# Autodesk Inventor assembly: Stator_Assembly_2_0_2
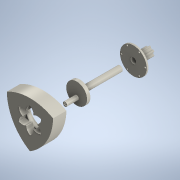
[picture p0: Inventor's stored thumbnail of the model, 180x180]
Saved by Autodesk Inventor 2021 (Build 250183000, 183)
## iProperties
Created: 2021-04-19
Part Number: Stator_Assembly_2_0_2
Document SubType Name: Assembly
Designer: lucia
Author: lucia
## Documents named in this file (4)
- E:\Documents\Inventor\Fixed Rotor Wankel Engine\Assemblies\Stator_Assembly_2_0_2.iam
- E:\Documents\Inventor\Fixed Rotor Wankel Engine\Parts\Rotor_Mount.ipt
- E:\Documents\Inventor\Fixed Rotor Wankel Engine\Parts\Eccentric_Shaft_2.ipt
- E:\Documents\Inventor\Fixed Rotor Wankel Engine\Parts\Rotor_Geared_6t_Mountable.ipt
## Components (3 placed, 3 different names)
1. Rotor_Mount:1 — Mate:1, Mate:2, Mate:3, Mate:4
2. Eccentric_Shaft_2:1 — Mate:3, Mate:4, Mate:5, Mate:6
3. Rotor_Geared_6t_Mountable:1 — Mate:5, Mate:6
## Relationships (6: Mate 6)
- Mate:1: Rotor_Mount:1
- Mate:2: Rotor_Mount:1
- Mate:3: Rotor_Mount:1 ↔ Eccentric_Shaft_2:1
- Mate:4 (203.2 mm): Rotor_Mount:1 ↔ Eccentric_Shaft_2:1
- Mate:5 (152.4 mm): Eccentric_Shaft_2:1 ↔ Rotor_Geared_6t_Mountable:1
- Mate:6: Eccentric_Shaft_2:1 ↔ Rotor_Geared_6t_Mountable:1
